# Autodesk Inventor assembly: 95648
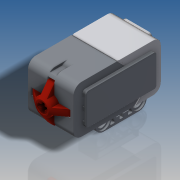
[picture p0: Inventor's stored thumbnail of the model, 180x180]
Saved by Autodesk Inventor 2016 SP2 (Build 200236200, 236)
## iProperties
Created: 2015-08-28
Part Number: 95648
Document SubType Name: Assembly
Designer: D. Kohfeld
Mass: 11.1928 g
Surface Area: 170.654 cm^2
Volume: 10.5592 cm^3
Density: 1.06 g/cm^3
Author: D. Kohfeld
## Documents named in this file (3)
- A:\LEGO Pieces\EV3\95648.iam
- A:\LEGO Pieces\EV3\99385c01.iam
- A:\LEGO Pieces\EV3\99386-Red.ipt
## Components (2 placed, 2 different names)
1. 99385c01:1 [sub-assembly] — Mate:1, Angle:1, Mate:2
2. 99386-Red:1 — Mate:1, Angle:1, Mate:2
## Relationships (3: Mate 2, Angle 1)
- Mate:1: 99385c01:1 ↔ 99386-Red:1
- Angle:1 (0 deg): 99385c01:1 ↔ 99386-Red:1
- Mate:2 (4 mm): 99385c01:1 ↔ 99386-Red:1
